# Autodesk Inventor assembly: Eslabon_RL
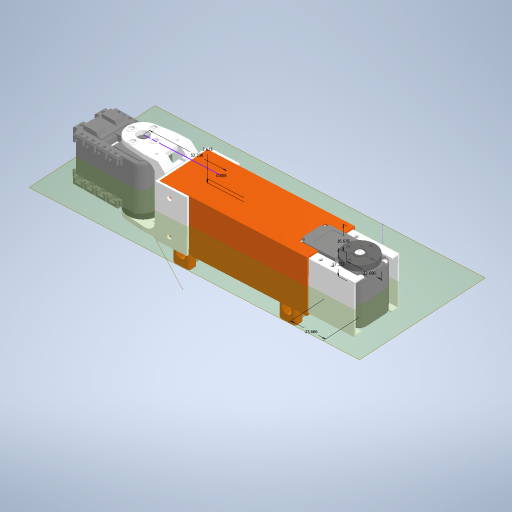
[picture p0: Inventor's stored thumbnail of the model, 512x512]
Saved by Autodesk Inventor 2024 (Build 280153000, 153)
## iProperties
Created: 2023-05-26
Part Number: Eslabon_RL
Document SubType Name: Assembly
Designer: epm01
Author: epm01
## Documents named in this file (5)
- D:\Archivos\Inventor\Adaptable\Eslabon_RL.iam
- D:\Archivos\Inventor\Adaptable\AX-12\AX-12.ipt
- D:\Archivos\Inventor\Adaptable\Eslabon_motor_R.iam
- D:\Archivos\Inventor\Adaptable\Eslabon_motor_L.iam
- D:\Archivos\Inventor\Adaptable\Polea.ipt
## Components (5 placed, 4 different names)
1. AX-12:1 — De rotación:1
2. Eslabon_motor_R:1 [sub-assembly] — De rotación:1, Coincidencia:1, Coincidencia:2, De rotación:2, De rotación:3, Corredera:1
3. Eslabon_motor_L:1 [sub-assembly] — Coincidencia:1, Coincidencia:2, Corredera:1
4. Polea:1 — De rotación:2
5. Polea:2 — De rotación:3
## Relationships (6: RevoluteJoint 3, Mate 2, TranslationJoint 1)
- De rotación:1 [RevoluteJoint]: AX-12:1 ↔ Eslabon_motor_R:1
- Coincidencia:1 [Mate]: Eslabon_motor_R:1 ↔ Eslabon_motor_L:1
- Coincidencia:2 [Mate]: Eslabon_motor_R:1 ↔ Eslabon_motor_L:1
- De rotación:2 [RevoluteJoint]: Eslabon_motor_R:1 ↔ Polea:1
- De rotación:3 [RevoluteJoint]: Eslabon_motor_R:1 ↔ Polea:2
- Corredera:1 [TranslationJoint]: Eslabon_motor_R:1 ↔ Eslabon_motor_L:1
